# Autodesk Inventor assembly: Panel_imitator
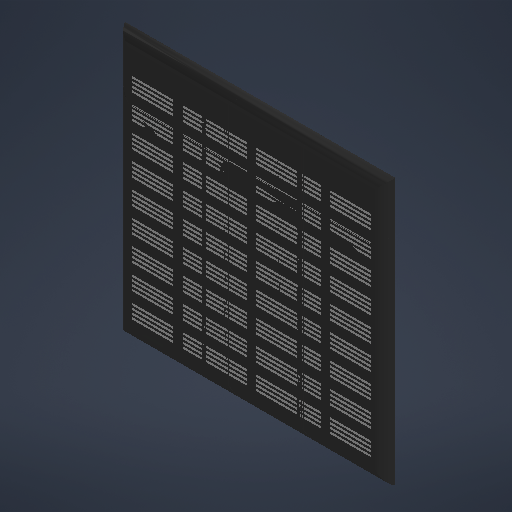
[picture p0: Inventor's stored thumbnail of the model, 512x512]
Saved by Autodesk Inventor 2027 (Build 310192060, 192F)
## iProperties
Created: 2026-05-30
Part Number: Panel_imitator
Document SubType Name: Assembly
Designer: User
Author: User
## Documents named in this file (2)
- C:\Users\Duszy\Desktop\Model\Panel_imitator.iam
- C:\Users\Duszy\Desktop\Model\SolarPanel_30x65x3mm.ipt
## Components (8 placed, 1 different names)
1. SolarPanel_30x65x3mm:1
2. SolarPanel_30x65x3mm:2
3. SolarPanel_30x65x3mm:3
4. SolarPanel_30x65x3mm:4
5. SolarPanel_30x65x3mm:5
6. SolarPanel_30x65x3mm:6
7. SolarPanel_30x65x3mm:7
8. SolarPanel_30x65x3mm:8
## Component patterns: (2 elements), (4 elements, first: SolarPanel_30x65x3mm:1), Szyk komponentów 1:2 (4 elements)
